# Autodesk Inventor assembly: WobbleGripper
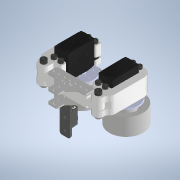
[picture p0: Inventor's stored thumbnail of the model, 180x180]
Saved by Autodesk Inventor 2021 (Build 250183000, 183)
## iProperties
Created: 2021-05-26
Part Number: WobbleGripper
Document SubType Name: Assembly
Designer: sami8
Author: sami8
## Documents named in this file (14)
- C:\Users\sami8\Documents\SGD-FTC2021\CAD\WobbleGripper.iam
- C:\Users\sami8\Documents\SGD-FTC2021\CAD\FloorRoller\REV-41-1097.ipt
- C:\Users\sami8\Documents\SGD-FTC2021\CAD\Shooter\REV-41-1125.ipt
- C:\Users\sami8\Documents\FTC 2021\CAD\Intake\REV-41-1846.ipt
- C:\Users\sami8\Documents\FTC 2021\CAD\Intake\am-3664 2in 5mm Hex Bore Stealth Wheel REV3.ipt
- C:\Users\sami8\Documents\SGD-FTC2021\CAD\FloorRoller\REV-41-1363.ipt
- C:\Users\sami8\Documents\SGD-FTC2021\CAD\WobbleGripper\M4x0.7_25mm_91290A176.ipt
- C:\Users\sami8\Documents\SGD-FTC2021\CAD\RearArm.ipt
- C:\Users\sami8\Documents\SGD-FTC2021\CAD\WobbleGripper\M5x0.8_30mm_91290A254.ipt
- C:\Users\sami8\Documents\SGD-FTC2021\CAD\WobbleGripper\M5x0.8mm_NYLOCK_90576A104.ipt
- C:\Users\sami8\Documents\SGD-FTC2021\CAD\WobbleGripper\REV-41-1483.ipt
- C:\Users\sami8\Documents\SGD-FTC2021\CAD\WobbleGripper\REV-31-1425.ipt
- C:\Users\sami8\Documents\SGD-FTC2021\CAD\ServoArm.iam
- C:\Users\sami8\Documents\SGD-FTC2021\CAD\ServoArm_MIR.iam
## Components (32 placed, 13 different names)
1. ServoArm:2 [sub-assembly] — Rigid:27, Rigid:28, Rigid:29, Rigid:30, Rigid:31, Rigid:32, Rigid:33, Mate:7, Mate:8, Angle:3, Mate:9
2. RearArm:1 — Rigid:25, Rigid:26, Rigid:27, Rigid:34
3. REV-41-1097:1 — Mate:7, Mate:8, Angle:3, Mate:9, Rigid:40
4. REV-41-1125:1 — Rigid:5
5. REV-41-1846:1 — Rigid:2, Rigid:3
6. am-3664 2in 5mm Hex Bore Stealth Wheel REV3:1 — Rigid:4, Rigid:5, Rigid:6
7. REV-41-1363:1 — Rigid:2, Rigid:40
8. REV-41-1846:2 — Rigid:3, Rigid:4
9. REV-41-1125:2 — Rigid:6
10. M4x0.7_25mm_91290A176:1 — Rigid:32
11. M4x0.7_25mm_91290A176:2 — Rigid:33
12. M4x0.7_25mm_91290A176:3 — Rigid:30
13. M4x0.7_25mm_91290A176:4 — Rigid:31
14. REV-41-1097:2 — Mate:10, Mate:11, Angle:4, Mate:12, Rigid:41
15. REV-41-1125:3
16. REV-41-1846:3
17. am-3664 2in 5mm Hex Bore Stealth Wheel REV3:2
18. REV-41-1363:2 — Rigid:41
19. REV-41-1846:4
20. REV-41-1125:4
21. M4x0.7_25mm_91290A176:5 — Rigid:35
22. M4x0.7_25mm_91290A176:6 — Rigid:36
23. M4x0.7_25mm_91290A176:7 — Rigid:39
24. M4x0.7_25mm_91290A176:8 — Rigid:38
25. M5x0.8_30mm_91290A254:1 — Rigid:28
26. M5x0.8mm_NYLOCK_90576A104:1 — Rigid:29
27. M5x0.8_30mm_91290A254:2 — Rigid:37
28. M5x0.8mm_NYLOCK_90576A104:2
29. REV-41-1483:1 — Rigid:25
30. REV-41-1483:2 — Rigid:26
31. REV-31-1425:1
32. ServoArm_MIR:1 [sub-assembly] — Rigid:34, Rigid:35, Rigid:36, Rigid:37, Rigid:38, Rigid:39, Mate:10, Mate:11, Angle:4, Mate:12
## Relationships (35: WeldJoint 27, Mate 6, Angle 2)
- Rigid:2 [WeldJoint]: REV-41-1846:1 ↔ REV-41-1363:1
- Rigid:3 [WeldJoint]: REV-41-1846:1 ↔ REV-41-1846:2
- Rigid:4 [WeldJoint]: am-3664 2in 5mm Hex Bore Stealth Wheel REV3:1 ↔ REV-41-1846:2
- Rigid:5 [WeldJoint]: REV-41-1125:1 ↔ am-3664 2in 5mm Hex Bore Stealth Wheel REV3:1
- Rigid:6 [WeldJoint]: am-3664 2in 5mm Hex Bore Stealth Wheel REV3:1 ↔ REV-41-1125:2
- [WeldJoint]: REV-41-1846:3 ↔ REV-41-1363:2
- [WeldJoint]: REV-41-1846:3 ↔ REV-41-1846:4
- [WeldJoint]: am-3664 2in 5mm Hex Bore Stealth Wheel REV3:2 ↔ REV-41-1846:4
- [WeldJoint]: REV-41-1125:3 ↔ am-3664 2in 5mm Hex Bore Stealth Wheel REV3:2
- [WeldJoint]: am-3664 2in 5mm Hex Bore Stealth Wheel REV3:2 ↔ REV-41-1125:4
- Rigid:25 [WeldJoint]: RearArm:1 ↔ REV-41-1483:1
- Rigid:26 [WeldJoint]: RearArm:1 ↔ REV-41-1483:2
- Rigid:27 [WeldJoint]: ServoArm:2 ↔ RearArm:1
- Rigid:28 [WeldJoint]: ServoArm:2 ↔ M5x0.8_30mm_91290A254:1
- Rigid:29 [WeldJoint]: ServoArm:2 ↔ M5x0.8mm_NYLOCK_90576A104:1
- Rigid:30 [WeldJoint]: ServoArm:2 ↔ M4x0.7_25mm_91290A176:3
- Rigid:31 [WeldJoint]: ServoArm:2 ↔ M4x0.7_25mm_91290A176:4
- Rigid:32 [WeldJoint]: ServoArm:2 ↔ M4x0.7_25mm_91290A176:1
- Rigid:33 [WeldJoint]: ServoArm:2 ↔ M4x0.7_25mm_91290A176:2
- Mate:7: ServoArm:2 ↔ REV-41-1097:1
- Mate:8: ServoArm:2 ↔ REV-41-1097:1
- Angle:3 (180.5 deg): ServoArm:2 ↔ REV-41-1097:1
- Mate:9 (1 mm): ServoArm:2 ↔ REV-41-1097:1
- Rigid:34 [WeldJoint]: RearArm:1 ↔ ServoArm_MIR:1
- Rigid:35 [WeldJoint]: M4x0.7_25mm_91290A176:5 ↔ ServoArm_MIR:1
- Rigid:36 [WeldJoint]: M4x0.7_25mm_91290A176:6 ↔ ServoArm_MIR:1
- Rigid:37 [WeldJoint]: M5x0.8_30mm_91290A254:2 ↔ ServoArm_MIR:1
- Rigid:38 [WeldJoint]: M4x0.7_25mm_91290A176:8 ↔ ServoArm_MIR:1
- Rigid:39 [WeldJoint]: M4x0.7_25mm_91290A176:7 ↔ ServoArm_MIR:1
- Mate:10: REV-41-1097:2 ↔ ServoArm_MIR:1
- Mate:11: REV-41-1097:2 ↔ ServoArm_MIR:1
- Angle:4 (179.5 deg): REV-41-1097:2 ↔ ServoArm_MIR:1
- Mate:12 (1 mm): REV-41-1097:2 ↔ ServoArm_MIR:1
- Rigid:40 [WeldJoint]: REV-41-1097:1 ↔ REV-41-1363:1
- Rigid:41 [WeldJoint]: REV-41-1097:2 ↔ REV-41-1363:2
## Named parameters: d15_d3 = 0 mm, d16_d4 = 0 mm, d17_d5 = 0 mm, d19_d1 = 0 mm, d20_d2 = 0 mm
